# Autodesk Inventor assembly: Gripper Attempt 02
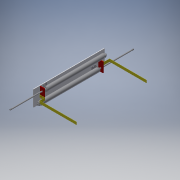
[picture p0: Inventor's stored thumbnail of the model, 180x180]
Saved by Autodesk Inventor 2016 (Build 200138000, 138)
## iProperties
Created: 2015-06-19
Part Number: Gripper Attempt 02
Document SubType Name: Assembly
Designer: steele
Author: steele
## Documents named in this file (8)
- C:\snobotics\CAD\robSteele\Gripper\Gripper Attempt 02.iam
- C:\snobotics\CAD\robSteele\ipart Components\Plate for Gripper\Plate for Gripper 6 x 27 x 1_4.ipt
- C:\snobotics\CAD\robSteele\ipart Components\Plate for Gripper.ipt
- C:\snobotics\CAD\partResources\McMaster-Carr\Air Cylinder\Pivot Mount Cylinders\Foot Bracket for 1_25 and 1_50 Bore\6498K340.ipt
- C:\snobotics\CAD\partResources\McMaster-Carr\Air Cylinder\Pivot Mount Cylinders\Single Acting With Spring Return\Force 155 Bore 1_50\Stroke 12\6498K786.ipt
- C:\snobotics\CAD\robSteele\ipart Components\Gripper Arm.ipt
- C:\snobotics\CAD\robSteele\ipart Components\Gripper Arm\Gripper Arm-02.ipt
- C:\snobotics\CAD\robSteele\Gripper\Gripper Piston.ipt
## Components (9 placed, 5 different names)
1. Plate for Gripper 6 x 27 x 1_4:1 — Mate:1, Flush:1, Flush:2, Mate:2, Flush:3, Flush:4, Flush:5, Mate:3
2. 6498K340:1 — Mate:2, Flush:3, Flush:4, Insert:2
3. 6498K340:2 — Mate:1, Flush:1, Flush:2, Insert:1
4. 6498K786:1 — Insert:1, Mate:4
5. 6498K786:2 — Insert:2, Insert:5
6. Gripper Arm-02:1 — Mate:6, Flush:8, Flush:9
7. Gripper Arm-02:2 — Mate:5, Flush:6, Flush:7
8. Gripper Piston:1 — Insert:5, Mate:5, Flush:6, Flush:7
9. Gripper Piston:2 — Flush:5, Mate:3, Mate:4, Mate:6, Flush:8, Flush:9
## Relationships (18: Flush 9, Mate 6, Insert 3)
- Mate:1: Plate for Gripper 6 x 27 x 1_4:1 ↔ 6498K340:2
- Flush:1: Plate for Gripper 6 x 27 x 1_4:1 ↔ 6498K340:2
- Flush:2 (558.8 mm): Plate for Gripper 6 x 27 x 1_4:1 ↔ 6498K340:2
- Mate:2: Plate for Gripper 6 x 27 x 1_4:1 ↔ 6498K340:1
- Flush:3: Plate for Gripper 6 x 27 x 1_4:1 ↔ 6498K340:1
- Flush:4 (558.8 mm): Plate for Gripper 6 x 27 x 1_4:1 ↔ 6498K340:1
- Insert:1: 6498K340:2 ↔ 6498K786:1
- Insert:2: 6498K340:1 ↔ 6498K786:2
- Insert:5 (12.7 mm): 6498K786:2 ↔ Gripper Piston:1
- Flush:5: Plate for Gripper 6 x 27 x 1_4:1 ↔ Gripper Piston:2
- Mate:3 (3.175 mm): Plate for Gripper 6 x 27 x 1_4:1 ↔ Gripper Piston:2
- Mate:4 (12.7 mm): 6498K786:1 ↔ Gripper Piston:2
- Mate:5: Gripper Arm-02:2 ↔ Gripper Piston:1
- Flush:6: Gripper Arm-02:2 ↔ Gripper Piston:1
- Flush:7: Gripper Arm-02:2 ↔ Gripper Piston:1
- Mate:6: Gripper Arm-02:1 ↔ Gripper Piston:2
- Flush:8: Gripper Arm-02:1 ↔ Gripper Piston:2
- Flush:9: Gripper Arm-02:1 ↔ Gripper Piston:2
## Named parameters: offsetToFrontOfAirCylinder = 558.8 mm
